# Autodesk Inventor assembly: 54
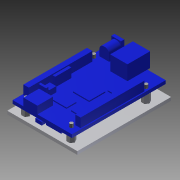
[picture p0: Inventor's stored thumbnail of the model, 180x180]
Saved by Autodesk Inventor 2013 (Build 170138000, 138)
## iProperties
Created: 2014-04-06
Part Number: 54
Document SubType Name: Assembly
Designer: andou
Author: andou
Title: CPU
## Documents named in this file (4)
- C:\Users\andou\Documents\GitHub\Robotics-Project\design\RoboticsProject\project_4\CPU.iam
- C:\Users\andou\Documents\GitHub\Robotics-Project\design\RoboticsProject\project_4\Generic Parts\Beagle_Bone_Black.ipt
- C:\Users\andou\Documents\GitHub\Robotics-Project\design\RoboticsProject\project_4\Beagle_Bone_Plate.ipt
- C:\Users\andou\Documents\GitHub\Robotics-Project\design\RoboticsProject\project_4\Generic Parts\Spacer(M3-8mm).ipt
## Components (6 placed, 3 different names)
1. Beagle_Bone_Black:1 — 挿入:1, 挿入:2, 挿入:3, 挿入:4
2. Beagle_Bone_Plate:1 — 挿入:5, 挿入:6
3. Spacer(M3-8mm):1 — 挿入:1, 挿入:5
4. Spacer(M3-8mm):2 — 挿入:2
5. Spacer(M3-8mm):3 — 挿入:4, 挿入:6
6. Spacer(M3-8mm):4 — 挿入:3
## Relationships (6: Insert 6)
- 挿入:1 [Insert]: Beagle_Bone_Black:1 ↔ Spacer(M3-8mm):1
- 挿入:2 [Insert]: Beagle_Bone_Black:1 ↔ Spacer(M3-8mm):2
- 挿入:3 [Insert]: Beagle_Bone_Black:1 ↔ Spacer(M3-8mm):4
- 挿入:4 [Insert]: Beagle_Bone_Black:1 ↔ Spacer(M3-8mm):3
- 挿入:5 [Insert]: Beagle_Bone_Plate:1 ↔ Spacer(M3-8mm):1
- 挿入:6 [Insert]: Beagle_Bone_Plate:1 ↔ Spacer(M3-8mm):3
